# Autodesk Inventor assembly: Silver
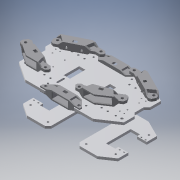
[picture p0: Inventor's stored thumbnail of the model, 180x180]
Saved by Autodesk Inventor 2016 (Build 200138000, 138)
## iProperties
Created: 2016-09-29
Part Number: Silver
Material: Générique
Document SubType Name: Assembly
Designer: LogOut
Author: LogOut
## Documents named in this file (9)
- C:\Travail\Objets\GitHub\Silver\Mechanic\Silver.iam
- C:\Travail\Objets\GitHub\Silver\Mechanic\Support_Roue.ipt
- C:\Travail\Objets\GitHub\Silver\Mechanic\Support_Moteur.ipt
- C:\Travail\Objets\GitHub\Silver\Mechanic\Support_GP2.C.ipt
- C:\Travail\Objets\GitHub\Silver\Mechanic\Support_GP2.Av.ipt
- C:\Travail\Objets\GitHub\Silver\Mechanic\Support_GP2.Ar.ipt
- C:\Travail\Objets\GitHub\Silver\Mechanic\Support_GP2.Av_MIR1.ipt
- C:\Travail\Objets\GitHub\Silver\Mechanic\Support_GP2.Ar_MIR2.ipt
- C:\Travail\Objets\GitHub\Silver\Mechanic\Support_GP2.C_MIR.ipt
## Components (9 placed, 8 different names)
1. Support_Roue:1 — Placage:2, Placage:13, Placage:14
2. Support_Roue:2 — Placage:1, Placage:11, Placage:12
3. Support_Moteur:1 — Placage:1, Placage:2, Placage:11, Placage:12, Placage:13, Placage:14, Placage:20, Placage:21, Placage:22, Placage:23, Placage:24
4. Support_GP2.C:1 — Placage:20, Placage:21, Placage:22, Placage:25
5. Support_GP2.Av:1 — Placage:23, Placage:24, Placage:25
6. Support_GP2.Ar:1
7. Support_GP2.Av_MIR1:1
8. Support_GP2.Ar_MIR2:1
9. Support_GP2.C_MIR:1
## Relationships (12: Mate 12)
- Placage:1 [Mate] (100 mm): Support_Roue:2 ↔ Support_Moteur:1
- Placage:2 [Mate] (100 mm): Support_Roue:1 ↔ Support_Moteur:1
- Placage:11 [Mate]: Support_Roue:2 ↔ Support_Moteur:1
- Placage:12 [Mate]: Support_Roue:2 ↔ Support_Moteur:1
- Placage:13 [Mate]: Support_Roue:1 ↔ Support_Moteur:1
- Placage:14 [Mate]: Support_Roue:1 ↔ Support_Moteur:1
- Placage:20 [Mate]: Support_Moteur:1 ↔ Support_GP2.C:1
- Placage:21 [Mate]: Support_Moteur:1 ↔ Support_GP2.C:1
- Placage:22 [Mate]: Support_Moteur:1 ↔ Support_GP2.C:1
- Placage:23 [Mate]: Support_Moteur:1 ↔ Support_GP2.Av:1
- Placage:24 [Mate]: Support_Moteur:1 ↔ Support_GP2.Av:1
- Placage:25 [Mate]: Support_GP2.C:1 ↔ Support_GP2.Av:1
